# Autodesk Inventor assembly: batt_MIR
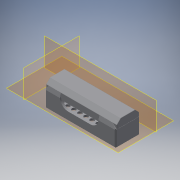
[picture p0: Inventor's stored thumbnail of the model, 180x180]
Saved by Autodesk Inventor 2016 (Build 200138000, 138)
## iProperties
Created: 2016-02-15
Part Number: batt_MIR
Document SubType Name: Assembly
Designer: jforce
Author: jforce
## Documents named in this file (3)
- C:\Users\jforce\Dropbox\gmu\ece590 (Selective Sync Conflict)\models3\batt_MIR.iam
- C:\Users\jforce\Dropbox\gmu\ece590 (Selective Sync Conflict)\models3\batt_cap_MIR.ipt
- C:\Users\jforce\Dropbox\gmu\ece590 (Selective Sync Conflict)\models3\batt_carrier_MIR.ipt
## Components (2 placed, 2 different names)
1. batt_cap_MIR:1 — Mate:2
2. batt_carrier_MIR:1 — Mate:2, Mate:1
## Relationships (2: Mate 2)
- Mate:2 (-6 mm): batt_cap_MIR:1 ↔ batt_carrier_MIR:1
- Mate:1: batt_carrier_MIR:1
